# Autodesk Inventor assembly: Ensamblaje asistente
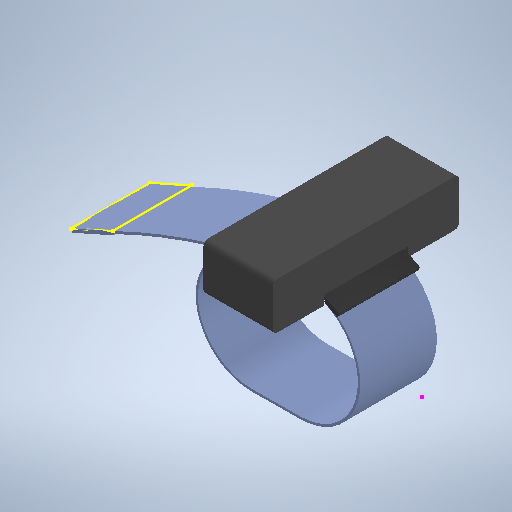
[picture p0: Inventor's stored thumbnail of the model, 512x512]
Saved by Autodesk Inventor 2025.2 (Build 292293000, 293)
## iProperties
Created: 2022-12-29
Part Number: Ensamblaje asistente
Document SubType Name: Assembly
Designer: asus
Sending System: SolidWorks 2021
Last Author: latti
Last Saved: 2022-12-31
Author: asus
## Documents named in this file (6)
- C:\Users\asus\Documents\Inventor\TFC\Ensamblaje asistente.iam
- C:\Users\asus\Documents\Inventor\TFC\cK watch\cK watch\cK watch strap clasp 1.ipt
- C:\Users\asus\Documents\Inventor\TFC\cK watch\cK watch\cK watch strap clasp 2.ipt
- C:\Users\asus\Documents\Inventor\TFC\Caja.ipt
- C:\Users\asus\Documents\Inventor\TFC\banda.ipt
- C:\Users\asus\Documents\Inventor\TFC\MAX30102EFD+T\MAX30102EFD+T\MAX30102EFD+T.ipt
## Components (5 placed, 5 different names)
1. cK watch strap clasp 1:1 — Insert:1, Mate:7
2. cK watch strap clasp 2:1 — Mate:1, Mate:2, Mate:3
3. Caja:1 — Insert:1, Mate:1, Mate:2, Mate:4, Mate:5, Mate:6
4. banda:1 — Mate:3, Mate:7
5. MAX30102EFD+T:1 — Mate:4, Mate:5, Mate:6
## Relationships (8: Mate 7, Insert 1)
- Insert:1: cK watch strap clasp 1:1 ↔ Caja:1
- Mate:1: cK watch strap clasp 2:1 ↔ Caja:1
- Mate:2 (0.2 mm): cK watch strap clasp 2:1 ↔ Caja:1
- Mate:3: cK watch strap clasp 2:1 ↔ banda:1
- Mate:4: Caja:1 ↔ MAX30102EFD+T:1
- Mate:5: Caja:1 ↔ MAX30102EFD+T:1
- Mate:6: Caja:1 ↔ MAX30102EFD+T:1
- Mate:7: cK watch strap clasp 1:1 ↔ banda:1
## Named parameters: Finish1_Area = 40.2205, Finish1_Thickness = 0.05 mm
note: some values were not read from the file. Shown as the stored number, unit unknown: "Finish1_Area".
